# Autodesk Inventor assembly: BaseEnsamble
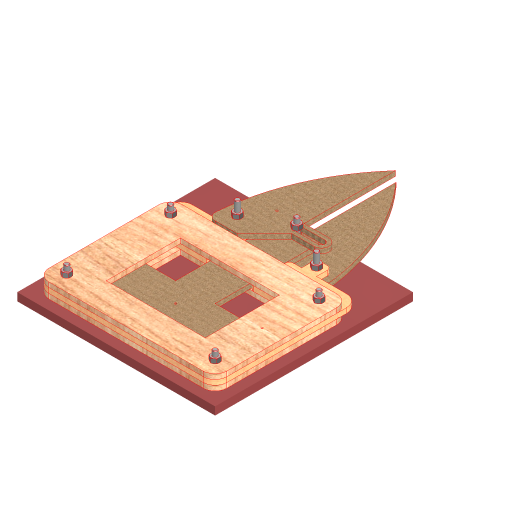
[picture p0: Inventor's stored thumbnail of the model, 512x512]
Saved by Autodesk Inventor 2023.2 (Build 272271000, 271)
## iProperties
Created: 2022-11-11
Part Number: BaseEnsamble
Document SubType Name: Assembly
Designer: Daniel Peña
Author: Daniel Peña
## Documents named in this file (4)
- E:\Daniel DiscoA\Documents\UNAL\ProyectoRobotica\CAD\V3 - BigChungus\BaseEnsamble.iam
- E:\Daniel DiscoA\Documents\UNAL\ProyectoRobotica\CAD\V3 - BigChungus\Piso.ipt
- E:\Daniel DiscoA\Documents\UNAL\ProyectoRobotica\CAD\V3 - BigChungus\Gripper General.iam
- E:\Daniel DiscoA\Documents\UNAL\ProyectoRobotica\CAD\V3 - BigChungus\PortaTornillos.ipt
## Components (3 placed, 3 different names)
1. Piso:1 — Flush:1
2. Gripper General:1 [sub-assembly] — Mate:1, Flush:2, Flush:3
3. PortaTornillos:1 — Flush:1, Mate:1, Flush:2, Flush:3
## Relationships (4: Flush 3, Mate 1)
- Flush:1: Piso:1 ↔ PortaTornillos:1
- Mate:1: Gripper General:1 ↔ PortaTornillos:1
- Flush:2 (10 mm): Gripper General:1 ↔ PortaTornillos:1
- Flush:3 (-10 mm): Gripper General:1 ↔ PortaTornillos:1
